# Autodesk Inventor assembly: Ethernet Switch Assembly
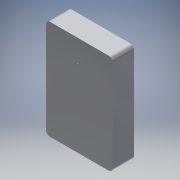
[picture p0: Inventor's stored thumbnail of the model, 180x180]
Saved by Autodesk Inventor 2017 (Build 210142000, 142)
## iProperties
Created: 2020-02-22
Part Number: Ethernet Switch Assembly
Document SubType Name: Assembly
Designer: S332848902
Author: S332848902
## Documents named in this file (3)
- \\ad.ocdsb.ca\studenthome\3\S338674153\FRC 2020\FullRobotRefactor\Parts\Ethernet Switch Assembly.iam
- \\ad.ocdsb.ca\studenthome\3\S338674153\FRC 2020\FullRobotRefactor\Parts\Ethernet switch.ipt
- \\ad.ocdsb.ca\studenthome\3\S338674153\FRC 2020\FullRobotRefactor\Parts\Ethernet Port.ipt
## Components (6 placed, 2 different names)
1. Ethernet switch:1 — Mate:1, Mate:2, Flush:1, Mate:3, Flush:2, Mate:5, Mate:6, Mate:7, Mate:9, Flush:3, Mate:10, Mate:12, Flush:4, Mate:13, Mate:14, Mate:15, Flush:5, Mate:16
2. Ethernet Port:1 — Mate:3, Mate:4, Flush:2, Mate:6, Mate:8
3. Ethernet Port:2 — Mate:10, Mate:11, Mate:12, Flush:4
4. Ethernet Port:3 — Mate:1, Mate:2, Flush:1, Mate:4, Mate:5
5. Ethernet Port:4 — Mate:13, Mate:14, Mate:15, Flush:5, Mate:16
6. Ethernet Port:5 — Mate:7, Mate:8, Mate:9, Flush:3, Mate:11
## Relationships (21: Mate 16, Flush 5)
- Mate:1: Ethernet switch:1 ↔ Ethernet Port:3
- Mate:2: Ethernet switch:1 ↔ Ethernet Port:3
- Flush:1: Ethernet switch:1 ↔ Ethernet Port:3
- Mate:3: Ethernet switch:1 ↔ Ethernet Port:1
- Mate:4: Ethernet Port:1 ↔ Ethernet Port:3
- Flush:2: Ethernet switch:1 ↔ Ethernet Port:1
- Mate:5: Ethernet switch:1 ↔ Ethernet Port:3
- Mate:6: Ethernet switch:1 ↔ Ethernet Port:1
- Mate:7: Ethernet switch:1 ↔ Ethernet Port:5
- Mate:8: Ethernet Port:1 ↔ Ethernet Port:5
- Mate:9: Ethernet switch:1 ↔ Ethernet Port:5
- Flush:3: Ethernet switch:1 ↔ Ethernet Port:5
- Mate:10: Ethernet switch:1 ↔ Ethernet Port:2
- Mate:11: Ethernet Port:2 ↔ Ethernet Port:5
- Mate:12: Ethernet switch:1 ↔ Ethernet Port:2
- Flush:4: Ethernet switch:1 ↔ Ethernet Port:2
- Mate:13: Ethernet switch:1 ↔ Ethernet Port:4
- Mate:14: Ethernet switch:1 ↔ Ethernet Port:4
- Mate:15: Ethernet switch:1 ↔ Ethernet Port:4
- Flush:5: Ethernet switch:1 ↔ Ethernet Port:4
- Mate:16: Ethernet switch:1 ↔ Ethernet Port:4
